# Autodesk Inventor assembly: MK5n, B (1)
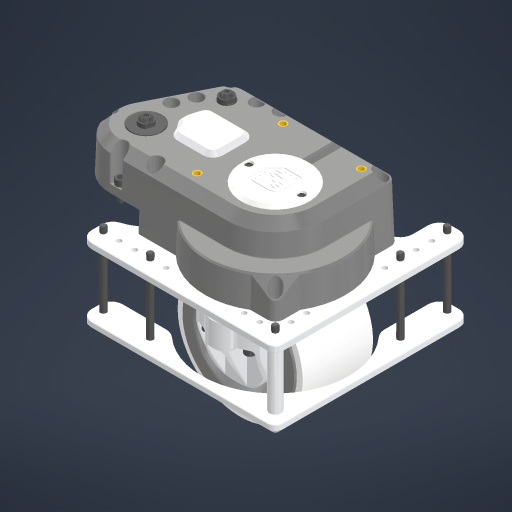
[picture p0: Inventor's stored thumbnail of the model, 512x512]
Saved by Autodesk Inventor 2024.4 (Build 284460000, 460)
## iProperties
Created: 2026-01-06
Part Number: MK5n, B (1)
Document SubType Name: Assembly
Designer: Kenji
Mass: 1769.01 g
Surface Area: 2127.48 cm^2
Volume: 1270.46 cm^3
Density: 1.39242 g/cm^3
Author: Kenji
Sending System: SOLIDWORKS 2022-2022290
MC: AMD64
MC_MODEL: Intel64 Family 6 Model 158 Stepping 10, GenuineIntel
OS: Windows_NT
FRU: Parasolid Version 33.1, build 260,  4-25-2022
FORMAT: text
GUISE: transmit
KEY: FILEMK5n, B.x_t
DATE: Fri Aug  8 12:41:37 2025
## Documents named in this file (11)
- C:\Users\Kenji\Documents\GitHub\1622-2026-Rebuilt\COTS Library\MK5n, B (1).iam
- C:\Users\Kenji\Downloads\MK5n, B (1)\MK5n, B (1)\MK5n, B (1).ipt
- C:\Users\Kenji\Downloads\MK5n, B (1)\MK5n, B (1)\MK5n, B (1)_1.ipt
- C:\Users\Kenji\Downloads\MK5n, B (1)\MK5n, B (1)\MK5n, B (1)_2.ipt
- C:\Users\Kenji\Downloads\MK5n, B (1)\MK5n, B (1)\MK5n, B (1)_3.ipt
- C:\Users\Kenji\Downloads\MK5n, B (1)\MK5n, B (1)\MK5n, B (1)_4.ipt
- C:\Users\Kenji\Downloads\MK5n, B (1)\MK5n, B (1)\MK5n, B (1)_5.ipt
- C:\Users\Kenji\Downloads\MK5n, B (1)\MK5n, B (1)\MK5n, B (1)_6.ipt
- C:\Users\Kenji\Downloads\MK5n, B (1)\MK5n, B (1)\MK5n, B (1)_7.ipt
- C:\Users\Kenji\Downloads\MK5n, B (1)\MK5n, B (1)\MK5n, B (1)_8.ipt
- C:\Users\Kenji\Downloads\MK5n, B (1)\MK5n, B (1)\MK5n, B (1)_9.ipt
## Components (10 placed, 10 different names)
1. MK5n, B (1) — Mate:10, Flush:1
2. MK5n, B (1)_1 — Mate:1, Mate:2, Mate:3, Mate:4
3. MK5n, B (1)_2 — Mate:14, Flush:2, Flush:3
4. MK5n, B (1)_3 — Mate:1, Mate:2, Angle:1
5. MK5n, B (1)_4 — Mate:13, Flush:3, Flush:4, Mate:15
6. MK5n, B (1)_5 — Mate:5, Mate:8, Mate:9, Mate:11, Mate:12, Mate:13, Mate:15
7. MK5n, B (1)_6 — Mate:6, Mate:7, Mate:8, Mate:9, Mate:14
8. MK5n, B (1)_7 — Mate:12, Flush:4
9. MK5n, B (1)_8 — Mate:11, Flush:1, Flush:2
10. MK5n, B (1)_9 — Mate:3, Mate:4, Angle:1, Mate:5, Mate:6, Mate:7, Mate:10, Angle:2
## Relationships (21: Mate 15, Flush 4, Angle 2)
- Mate:1: MK5n, B (1)_1 ↔ MK5n, B (1)_3
- Mate:2: MK5n, B (1)_1 ↔ MK5n, B (1)_3
- Mate:3: MK5n, B (1)_1 ↔ MK5n, B (1)_9
- Mate:4: MK5n, B (1)_1 ↔ MK5n, B (1)_9
- Angle:1 (0 deg): MK5n, B (1)_3 ↔ MK5n, B (1)_9
- Mate:5: MK5n, B (1)_5 ↔ MK5n, B (1)_9
- Mate:6: MK5n, B (1)_6 ↔ MK5n, B (1)_9
- Mate:7: MK5n, B (1)_6 ↔ MK5n, B (1)_9
- Mate:8: MK5n, B (1)_5 ↔ MK5n, B (1)_6
- Mate:9: MK5n, B (1)_5 ↔ MK5n, B (1)_6
- Mate:10: MK5n, B (1) ↔ MK5n, B (1)_9
- Mate:11: MK5n, B (1)_5 ↔ MK5n, B (1)_8
- Mate:12: MK5n, B (1)_5 ↔ MK5n, B (1)_7
- Mate:13: MK5n, B (1)_4 ↔ MK5n, B (1)_5
- Mate:14: MK5n, B (1)_2 ↔ MK5n, B (1)_6
- Flush:1: MK5n, B (1) ↔ MK5n, B (1)_8
- Flush:2: MK5n, B (1)_2 ↔ MK5n, B (1)_8
- Flush:3: MK5n, B (1)_2 ↔ MK5n, B (1)_4
- Flush:4: MK5n, B (1)_4 ↔ MK5n, B (1)_7
- Mate:15: MK5n, B (1)_4 ↔ MK5n, B (1)_5
- Angle:2 (0 deg): MK5n, B (1)_9
